# Autodesk Inventor assembly: Robot Arm mods
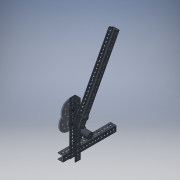
[picture p0: Inventor's stored thumbnail of the model, 180x180]
Saved by Autodesk Inventor 2016 (Build 200138000, 138)
## iProperties
Created: 2015-12-15
Part Number: Robot Arm mods
Document SubType Name: Assembly
Designer: tbloo
Author: tbloo
## Documents named in this file (11)
- C:\Users\tbloo\Documents\GitHub\phi_robotics\3d-models\FTC_Tetrix_KOP_Block_Party\Tim Bloot Designs\JAr JaR Bot\Robot Arm mods.iam
- C:\Users\tbloo\Documents\GitHub\phi_robotics\3d-models\FTC_Tetrix_KOP_Block_Party\Tetrix_Kit_FTC\Autodesk Inventor Files\tetrix_c_channel-4.ipt
- C:\Users\tbloo\Documents\GitHub\phi_robotics\3d-models\FTC_Tetrix_KOP_Block_Party\Tetrix_Kit_FTC\Autodesk Inventor Files\tetrix_c_channel-5.ipt
- C:\Users\tbloo\Documents\GitHub\phi_robotics\3d-models\FTC_Tetrix_KOP_Block_Party\Tetrix_Kit_FTC\Autodesk Inventor Files\tetrix_gear-small.ipt
- C:\Users\tbloo\Documents\GitHub\phi_robotics\3d-models\FTC_Tetrix_KOP_Block_Party\Tetrix_Kit_FTC\Autodesk Inventor Files\tetrix_gear-large.ipt
- C:\Users\tbloo\Documents\GitHub\phi_robotics\3d-models\FTC_Tetrix_KOP_Block_Party\Tetrix_Kit_FTC\Autodesk Inventor Files\tetrix_bushing.ipt
- C:\Users\tbloo\Documents\GitHub\phi_robotics\3d-models\FTC_Tetrix_KOP_Block_Party\Tetrix_Kit_FTC\Autodesk Inventor Files\tetrix_axle.ipt
- C:\Users\tbloo\Documents\GitHub\phi_robotics\3d-models\FTC_Tetrix_KOP_Block_Party\Tetrix_Kit_FTC\Autodesk Inventor Files\tetrix_axle_lock.iam
- C:\Users\tbloo\Documents\GitHub\phi_robotics\3d-models\FTC_Tetrix_KOP_Block_Party\Tetrix_Kit_FTC\Autodesk Inventor Files\tetrix_739092_2012.iam
- C:\Users\tbloo\Documents\GitHub\phi_robotics\3d-models\FTC_Tetrix_KOP_Block_Party\Tetrix_Kit_FTC\Autodesk Inventor Files\tetrix_motor_mount-old.ipt
- C:\Users\tbloo\Documents\GitHub\phi_robotics\3d-models\FTC_Tetrix_KOP_Block_Party\Tetrix_Kit_FTC\Autodesk Inventor Files\tetrix_motor.iam
## Components (21 placed, 10 different names)
1. tetrix_c_channel-4:2 — Rigid:1
2. tetrix_c_channel-4:3 — Rigid:1, Rotational:1, Rotational:2, Rotational:4, Rotational:5, Rigid:14
3. tetrix_c_channel-5:1 — Rigid:2, Rigid:4
4. tetrix_gear-small:1
5. tetrix_gear-small:2 — Rigid:10, Rigid:13
6. tetrix_gear-large:1 — Rigid:5
7. tetrix_gear-large:2 — Rigid:12
8. tetrix_bushing:1 — Rotational:2, Rigid:7
9. tetrix_bushing:2 — Rotational:1
10. tetrix_bushing:3 — Rotational:5, Rigid:11
11. tetrix_bushing:4 — Rotational:3, Rotational:4
12. tetrix_axle:1 — Rigid:9
13. tetrix_axle:2 — Rigid:3, Rigid:8
14. tetrix_axle_lock:1 [sub-assembly] — Rigid:2, Rigid:3
15. tetrix_axle_lock:2 [sub-assembly] — Rigid:4, Rigid:7
16. tetrix_axle_lock:3 [sub-assembly] — Rigid:5, Rigid:8
17. tetrix_739092_2012:1 [sub-assembly] — Rigid:9, Rotational:3
18. tetrix_axle_lock:4 [sub-assembly] — Rigid:10, Rigid:11
19. tetrix_axle_lock:5 [sub-assembly] — Rigid:12, Rigid:13
20. tetrix_motor_mount-old:1 — Rigid:14, Rotational:6
21. tetrix_motor:1 [sub-assembly] — Rotational:6
## Relationships (19: WeldJoint 13, RevoluteJoint 6)
- Rigid:1 [WeldJoint]: tetrix_c_channel-4:2 ↔ tetrix_c_channel-4:3
- Rotational:1 [RevoluteJoint]: tetrix_c_channel-4:3 ↔ tetrix_bushing:2
- Rotational:2 [RevoluteJoint]: tetrix_c_channel-4:3 ↔ tetrix_bushing:1
- Rigid:2 [WeldJoint]: tetrix_c_channel-5:1 ↔ tetrix_axle_lock:1
- Rigid:3 [WeldJoint]: tetrix_axle:2 ↔ tetrix_axle_lock:1
- Rigid:4 [WeldJoint]: tetrix_c_channel-5:1 ↔ tetrix_axle_lock:2
- Rigid:7 [WeldJoint]: tetrix_bushing:1 ↔ tetrix_axle_lock:2
- Rigid:5 [WeldJoint]: tetrix_gear-large:1 ↔ tetrix_axle_lock:3
- Rigid:8 [WeldJoint] (19.3 mm): tetrix_axle:2 ↔ tetrix_axle_lock:3
- Rigid:9 [WeldJoint]: tetrix_axle:1 ↔ tetrix_739092_2012:1
- Rotational:3 [RevoluteJoint]: tetrix_bushing:4 ↔ tetrix_739092_2012:1
- Rotational:4 [RevoluteJoint]: tetrix_c_channel-4:3 ↔ tetrix_bushing:4
- Rotational:5 [RevoluteJoint]: tetrix_c_channel-4:3 ↔ tetrix_bushing:3
- Rigid:10 [WeldJoint]: tetrix_gear-small:2 ↔ tetrix_axle_lock:4
- Rigid:11 [WeldJoint]: tetrix_bushing:3 ↔ tetrix_axle_lock:4
- Rigid:12 [WeldJoint]: tetrix_gear-large:2 ↔ tetrix_axle_lock:5
- Rigid:13 [WeldJoint]: tetrix_gear-small:2 ↔ tetrix_axle_lock:5
- Rigid:14 [WeldJoint]: tetrix_c_channel-4:3 ↔ tetrix_motor_mount-old:1
- Rotational:6 [RevoluteJoint]: tetrix_motor_mount-old:1 ↔ tetrix_motor:1
